# Autodesk Inventor assembly: HUB CENTER
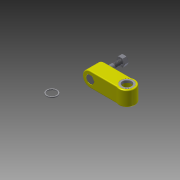
[picture p0: Inventor's stored thumbnail of the model, 180x180]
Saved by Autodesk Inventor 2013 (Build 170138000, 138)
## iProperties
Created: 2013-11-26
Part Number: HUB CENTER
Document SubType Name: Assembly
Designer: employee
Author: employee
## Documents named in this file (7)
- C:\Users\employee\Desktop\ConceptFORGE\ConceptFORGE\GUS Simpson\INVENTOR FILES\HUB CENTER.iam
- C:\Users\employee\Desktop\ConceptFORGE\ConceptFORGE\GUS Simpson\INVENTOR FILES\HUB CENTER.ipt
- C:\Users\employee\Desktop\ConceptFORGE\ConceptFORGE\GUS Simpson\INVENTOR FILES\M8x55.ipt
- C:\Users\employee\Desktop\ConceptFORGE\ConceptFORGE\GUS Simpson\INVENTOR FILES\M8 NUT.ipt
- C:\Users\employee\Desktop\ConceptFORGE\ConceptFORGE\GUS Simpson\INVENTOR FILES\M8 WASHER.ipt
- C:\Users\employee\Desktop\ConceptFORGE\ConceptFORGE\GUS Simpson\INVENTOR FILES\_6702.ipt
- C:\Users\employee\Desktop\ConceptFORGE\ConceptFORGE\GUS Simpson\INVENTOR FILES\HUB WASHER.ipt
## Components (7 placed, 6 different names)
1. HUB CENTER:1 — Insert:1, Angle:1, Insert:2, Insert:4, Insert:5
2. M8x55:1 — Insert:1, Angle:1
3. M8 NUT:1 — Insert:3
4. M8 WASHER:1 — Insert:2, Insert:3
5. _6702:1 — Insert:4, Insert:6
6. _6702:2 — Insert:5
7. HUB WASHER:1 — Insert:6
## Relationships (7: Insert 6, Angle 1)
- Insert:1: HUB CENTER:1 ↔ M8x55:1
- Angle:1 (0 deg): HUB CENTER:1 ↔ M8x55:1
- Insert:2: HUB CENTER:1 ↔ M8 WASHER:1
- Insert:3 (25 mm): M8 NUT:1 ↔ M8 WASHER:1
- Insert:4: HUB CENTER:1 ↔ _6702:1
- Insert:5: HUB CENTER:1 ↔ _6702:2
- Insert:6: _6702:1 ↔ HUB WASHER:1
